# Autodesk Inventor assembly: Nut-M4-2021
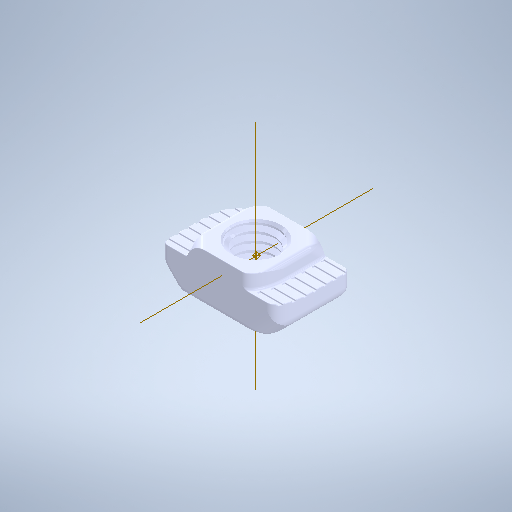
[picture p0: Inventor's stored thumbnail of the model, 512x512]
Saved by Autodesk Inventor 2025 (Build 290162000, 162)
## iProperties
Created: 2025-10-11
Part Number: Nut-M4-2021
Document SubType Name: Assembly
Designer: hp
Author: hp
## Documents named in this file (2)
- D:\gp amr\nut-m4-2020-10-6mm-1.snapshot.6\Nut-M4-2020\Nut-M4-2021.iam
- D:\gp amr\nut-m4-2020-10-6mm-1.snapshot.6\Nut-M4-2020\Nut-M4-2020.ipt
## Components (1 placed, 1 different names)
1. Nut-M4-2020:1 — Mate:1, Mate:2
## Relationships (2: Mate 2)
- Mate:1: Nut-M4-2020:1
- Mate:2: Nut-M4-2020:1
